# Autodesk Inventor assembly: Motor arm assembly
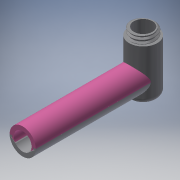
[picture p0: Inventor's stored thumbnail of the model, 180x180]
Saved by Autodesk Inventor 2019 (Build 230136000, 136)
## iProperties
Created: 2020-03-26
Part Number: Motor arm assembly
Document SubType Name: Assembly
Designer: 18186
Author: 18186
## Documents named in this file (3)
- D:\CoDrone\Motor arm assembly.iam
- D:\CoDrone\drone motor arm bottom.ipt
- D:\CoDrone\drone motor arm top.ipt
## Components (2 placed, 2 different names)
1. drone motor arm bottom:1 — Mate:1, Flush:1
2. drone motor arm top:1 — Mate:1, Flush:1
## Relationships (2: Mate 1, Flush 1)
- Mate:1: drone motor arm bottom:1 ↔ drone motor arm top:1
- Flush:1: drone motor arm bottom:1 ↔ drone motor arm top:1
